# Autodesk Inventor assembly: 혼축링크
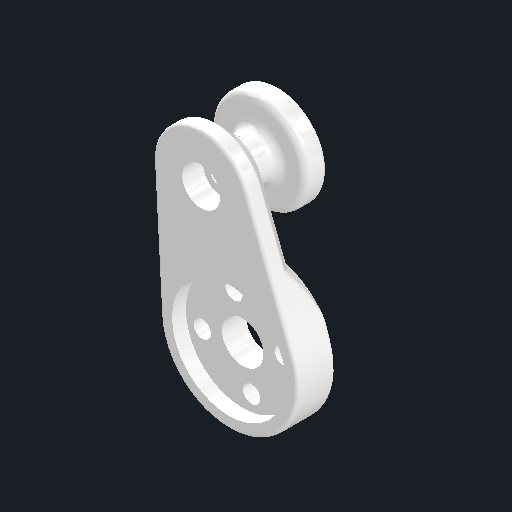
[picture p0: Inventor's stored thumbnail of the model, 512x512]
Saved by Autodesk Inventor 2027.1 (Build 311270010, 270A)
## iProperties
Created: 2026-08-22
Part Number: 혼축링크
Document SubType Name: Assembly
Designer: moieboy9999
Mass: 2.60074 g
Surface Area: 22.6438 cm^2
Volume: 2.45353 cm^3
Density: 1.06 g/cm^3
Author: moieboy9999
## Documents named in this file (3)
- D:\micro_dog_cad\다리\프레임\혼축링크.iam
- D:\micro_dog_cad\다리\프레임\링크축.ipt
- D:\micro_dog_cad\다리\프레임\링크 고정.ipt
## Components (2 placed, 2 different names)
1. 링크축:1
2. 링크 고정:1
## Relationships (2: Mate 2)
- [Mate]: 링크축:1 ↔ 링크 고정:1
- [Mate]: 링크축:1 ↔ 링크 고정:1
